# Autodesk Inventor assembly: Frame 1771926384246
(part 2 of 3)
- C:\Users\Admin01\Documents\WU15\TRASTRGNN\Inventor\StructureGenerator\Frame\ANSI UP8 x 30 1771926400178.ipt
- C:\Users\Admin01\Documents\WU15\TRASTRGNN\Inventor\StructureGenerator\Frame\ANSI UP8 x 30 1771926400208.ipt
- C:\Users\Admin01\Documents\WU15\TRASTRGNN\Inventor\StructureGenerator\Frame\ANSI UP8 x 30 1771926400238.ipt
- C:\Users\Admin01\Documents\WU15\TRASTRGNN\Inventor\StructureGenerator\Frame\ANSI UP8 x 30 1771926400267.ipt
- C:\Users\Admin01\Documents\WU15\TRASTRGNN\Inventor\StructureGenerator\Frame\ANSI UP8 x 30 1771926400297.ipt
- C:\Users\Admin01\Documents\WU15\TRASTRGNN\Inventor\StructureGenerator\Frame\ANSI UP8 x 30 1771926400327.ipt
- C:\Users\Admin01\Documents\WU15\TRASTRGNN\Inventor\StructureGenerator\Frame\ANSI UP8 x 30 1771926400356.ipt
- C:\Users\Admin01\Documents\WU15\TRASTRGNN\Inventor\StructureGenerator\Frame\ANSI UP8 x 30 1771926400385.ipt
- C:\Users\Admin01\Documents\WU15\TRASTRGNN\Inventor\StructureGenerator\Frame\ANSI UP8 x 30 1771926400415.ipt
- C:\Users\Admin01\Documents\WU15\TRASTRGNN\Inventor\StructureGenerator\Frame\ANSI UP8 x 30 1771926400444.ipt
- C:\Users\Admin01\Documents\WU15\TRASTRGNN\Inventor\StructureGenerator\Frame\ANSI UP8 x 30 1771926400474.ipt
- C:\Users\Admin01\Documents\WU15\TRASTRGNN\Inventor\StructureGenerator\Frame\ANSI UP8 x 30 1771926400503.ipt
- C:\Users\Admin01\Documents\WU15\TRASTRGNN\Inventor\StructureGenerator\Frame\ANSI UP8 x 30 1771926400533.ipt
- C:\Users\Admin01\Documents\WU15\TRASTRGNN\Inventor\StructureGenerator\Frame\ANSI UP8 x 30 1771926400563.ipt
- C:\Users\Admin01\Documents\WU15\TRASTRGNN\Inventor\StructureGenerator\Frame\ANSI UP8 x 30 1771926400592.ipt
- C:\Users\Admin01\Documents\WU15\TRASTRGNN\Inventor\StructureGenerator\Frame\ANSI UP8 x 30 1771926400622.ipt
- C:\Users\Admin01\Documents\WU15\TRASTRGNN\Inventor\StructureGenerator\Frame\ANSI UP8 x 30 1771926400652.ipt
- C:\Users\Admin01\Documents\WU15\TRASTRGNN\Inventor\StructureGenerator\Frame\ANSI UP8 x 30 1771926400682.ipt
- C:\Users\Admin01\Documents\WU15\TRASTRGNN\Inventor\StructureGenerator\Frame\ANSI UP8 x 30 1771926400712.ipt
- C:\Users\Admin01\Documents\WU15\TRASTRGNN\Inventor\StructureGenerator\Frame\ANSI UP8 x 30 1771926400742.ipt
- C:\Users\Admin01\Documents\WU15\TRASTRGNN\Inventor\StructureGenerator\Frame\ANSI UP8 x 30 1771926400772.ipt
- C:\Users\Admin01\Documents\WU15\TRASTRGNN\Inventor\StructureGenerator\Frame\ANSI UP8 x 30 1771926400801.ipt
- C:\Users\Admin01\Documents\WU15\TRASTRGNN\Inventor\StructureGenerator\Frame\ANSI UP8 x 30 1771926400831.ipt
- C:\Users\Admin01\Documents\WU15\TRASTRGNN\Inventor\StructureGenerator\Frame\ANSI UP8 x 30 1771926400861.ipt
- C:\Users\Admin01\Documents\WU15\TRASTRGNN\Inventor\StructureGenerator\Frame\ANSI UP8 x 30 1771926400890.ipt
- C:\Users\Admin01\Documents\WU15\TRASTRGNN\Inventor\StructureGenerator\Frame\ANSI UP8 x 30 1771926400920.ipt
- C:\Users\Admin01\Documents\WU15\TRASTRGNN\Inventor\StructureGenerator\Frame\ANSI UP8 x 30 1771926400949.ipt
- C:\Users\Admin01\Documents\WU15\TRASTRGNN\Inventor\StructureGenerator\Frame\ANSI UP8 x 30 1771926400979.ipt
- C:\Users\Admin01\Documents\WU15\TRASTRGNN\Inventor\StructureGenerator\Frame\ANSI UP8 x 30 1771926401008.ipt
- C:\Users\Admin01\Documents\WU15\TRASTRGNN\Inventor\StructureGenerator\Frame\ANSI UP8 x 30 1771926401039.ipt
- C:\Users\Admin01\Documents\WU15\TRASTRGNN\Inventor\StructureGenerator\Frame\ANSI UP8 x 30 1771926401068.ipt
- C:\Users\Admin01\Documents\WU15\TRASTRGNN\Inventor\StructureGenerator\Frame\ANSI UP8 x 30 1771926401100.ipt
- C:\Users\Admin01\Documents\WU15\TRASTRGNN\Inventor\StructureGenerator\Frame\ANSI UP8 x 30 1771926401129.ipt
- C:\Users\Admin01\Documents\WU15\TRASTRGNN\Inventor\StructureGenerator\Frame\ANSI UP8 x 30 1771926401159.ipt
- C:\Users\Admin01\Documents\WU15\TRASTRGNN\Inventor\StructureGenerator\Frame\ANSI UP8 x 30 1771926401189.ipt
- C:\Users\Admin01\Documents\WU15\TRASTRGNN\Inventor\StructureGenerator\Frame\ANSI UP8 x 30 1771926401219.ipt
- C:\Users\Admin01\Documents\WU15\TRASTRGNN\Inventor\StructureGenerator\Frame\ANSI UP8 x 30 1771926401248.ipt
- C:\Users\Admin01\Documents\WU15\TRASTRGNN\Inventor\StructureGenerator\Frame\ANSI UP8 x 30 1771926401278.ipt
- C:\Users\Admin01\Documents\WU15\TRASTRGNN\Inventor\StructureGenerator\Frame\ANSI UP8 x 30 1771926401307.ipt
- C:\Users\Admin01\Documents\WU15\TRASTRGNN\Inventor\StructureGenerator\Frame\ANSI UP8 x 30 1771926401337.ipt
- C:\Users\Admin01\Documents\WU15\TRASTRGNN\Inventor\StructureGenerator\Frame\ANSI UP8 x 30 1771926401367.ipt
- C:\Users\Admin01\Documents\WU15\TRASTRGNN\Inventor\StructureGenerator\Frame\ANSI UP8 x 30 1771926401396.ipt
- C:\Users\Admin01\Documents\WU15\TRASTRGNN\Inventor\StructureGenerator\Frame\ANSI UP8 x 30 1771926401425.ipt
- C:\Users\Admin01\Documents\WU15\TRASTRGNN\Inventor\StructureGenerator\Frame\ANSI UP8 x 30 1771926401455.ipt
- C:\Users\Admin01\Documents\WU15\TRASTRGNN\Inventor\StructureGenerator\Frame\ANSI UP8 x 30 1771926401488.ipt
- C:\Users\Admin01\Documents\WU15\TRASTRGNN\Inventor\StructureGenerator\Frame\ANSI UP8 x 30 1771926401519.ipt
- C:\Users\Admin01\Documents\WU15\TRASTRGNN\Inventor\StructureGenerator\Frame\ANSI UP8 x 30 1771926401550.ipt
- C:\Users\Admin01\Documents\WU15\TRASTRGNN\Inventor\StructureGenerator\Frame\ANSI UP8 x 30 1771926401585.ipt
- C:\Users\Admin01\Documents\WU15\TRASTRGNN\Inventor\StructureGenerator\Frame\ANSI UP8 x 30 1771926401618.ipt
- C:\Users\Admin01\Documents\WU15\TRASTRGNN\Inventor\StructureGenerator\Frame\ANSI UP8 x 30 1771926401651.ipt
- C:\Users\Admin01\Documents\WU15\TRASTRGNN\Inventor\StructureGenerator\Frame\ANSI UP8 x 30 1771926401685.ipt
- C:\Users\Admin01\Documents\WU15\TRASTRGNN\Inventor\StructureGenerator\Frame\ANSI UP8 x 30 1771926401716.ipt
- C:\Users\Admin01\Documents\WU15\TRASTRGNN\Inventor\StructureGenerator\Frame\ANSI UP8 x 30 1771926401746.ipt
- C:\Users\Admin01\Documents\WU15\TRASTRGNN\Inventor\StructureGenerator\Frame\ANSI UP8 x 30 1771926401775.ipt
- C:\Users\Admin01\Documents\WU15\TRASTRGNN\Inventor\StructureGenerator\Frame\ANSI UP8 x 30 1771926401805.ipt
- C:\Users\Admin01\Documents\WU15\TRASTRGNN\Inventor\StructureGenerator\Frame\ANSI UP8 x 30 1771926401837.ipt
- C:\Users\Admin01\Documents\WU15\TRASTRGNN\Inventor\StructureGenerator\Frame\ANSI UP8 x 30 1771926401868.ipt
- C:\Users\Admin01\Documents\WU15\TRASTRGNN\Inventor\StructureGenerator\Frame\ANSI UP8 x 30 1771926401898.ipt
- C:\Users\Admin01\Documents\WU15\TRASTRGNN\Inventor\StructureGenerator\Frame\ANSI UP8 x 30 1771926401929.ipt
- C:\Users\Admin01\Documents\WU15\TRASTRGNN\Inventor\StructureGenerator\Frame\ANSI UP8 x 30 1771926401960.ipt
- C:\Users\Admin01\Documents\WU15\TRASTRGNN\Inventor\StructureGenerator\Frame\ANSI UP8 x 30 1771926401992.ipt
- C:\Users\Admin01\Documents\WU15\TRASTRGNN\Inventor\StructureGenerator\Frame\ANSI UP8 x 30 1771926402023.ipt
- C:\Users\Admin01\Documents\WU15\TRASTRGNN\Inventor\StructureGenerator\Frame\ANSI UP8 x 30 1771926402053.ipt
- C:\Users\Admin01\Documents\WU15\TRASTRGNN\Inventor\StructureGenerator\Frame\ANSI UP8 x 30 1771926402084.ipt
- C:\Users\Admin01\Documents\WU15\TRASTRGNN\Inventor\StructureGenerator\Frame\ANSI UP8 x 30 1771926402116.ipt
- C:\Users\Admin01\Documents\WU15\TRASTRGNN\Inventor\StructureGenerator\Frame\ANSI UP8 x 30 1771926402147.ipt
- C:\Users\Admin01\Documents\WU15\TRASTRGNN\Inventor\StructureGenerator\Frame\ANSI UP8 x 30 1771926402182.ipt
- C:\Users\Admin01\Documents\WU15\TRASTRGNN\Inventor\StructureGenerator\Frame\ANSI UP8 x 30 1771926402214.ipt
- C:\Users\Admin01\Documents\WU15\TRASTRGNN\Inventor\StructureGenerator\Frame\ANSI UP8 x 30 1771926402248.ipt
- C:\Users\Admin01\Documents\WU15\TRASTRGNN\Inventor\StructureGenerator\Frame\ANSI UP8 x 30 1771926402278.ipt
- C:\Users\Admin01\Documents\WU15\TRASTRGNN\Inventor\StructureGenerator\Frame\ANSI UP8 x 30 1771926402309.ipt
- C:\Users\Admin01\Documents\WU15\TRASTRGNN\Inventor\StructureGenerator\Frame\ANSI UP8 x 30 1771926402354.ipt
- C:\Users\Admin01\Documents\WU15\TRASTRGNN\Inventor\StructureGenerator\Frame\ANSI UP8 x 30 1771926402386.ipt
- C:\Users\Admin01\Documents\WU15\TRASTRGNN\Inventor\StructureGenerator\Frame\ANSI UP8 x 30 1771926402418.ipt
- C:\Users\Admin01\Documents\WU15\TRASTRGNN\Inventor\StructureGenerator\Frame\ANSI UP8 x 30 1771926402453.ipt
- C:\Users\Admin01\Documents\WU15\TRASTRGNN\Inventor\StructureGenerator\Frame\ANSI UP8 x 30 1771926402485.ipt
- C:\Users\Admin01\Documents\WU15\TRASTRGNN\Inventor\StructureGenerator\Frame\ANSI UP8 x 30 1771926402516.ipt
- C:\Users\Admin01\Documents\WU15\TRASTRGNN\Inventor\StructureGenerator\Frame\ANSI UP8 x 30 1771926402546.ipt
- C:\Users\Admin01\Documents\WU15\TRASTRGNN\Inventor\StructureGenerator\Frame\ANSI UP8 x 30 1771926402576.ipt
- C:\Users\Admin01\Documents\WU15\TRASTRGNN\Inventor\StructureGenerator\Frame\ANSI UP8 x 30 1771926402607.ipt
- C:\Users\Admin01\Documents\WU15\TRASTRGNN\Inventor\StructureGenerator\Frame\ANSI UP8 x 30 1771926402637.ipt
- C:\Users\Admin01\Documents\WU15\TRASTRGNN\Inventor\StructureGenerator\Frame\ANSI UP8 x 30 1771926402667.ipt
- C:\Users\Admin01\Documents\WU15\TRASTRGNN\Inventor\StructureGenerator\Frame\ANSI UP8 x 30 1771926402697.ipt
- C:\Users\Admin01\Documents\WU15\TRASTRGNN\Inventor\StructureGenerator\Frame\ANSI UP8 x 30 1771926402726.ipt
- C:\Users\Admin01\Documents\WU15\TRASTRGNN\Inventor\StructureGenerator\Frame\ANSI UP8 x 30 1771926402756.ipt
- C:\Users\Admin01\Documents\WU15\TRASTRGNN\Inventor\StructureGenerator\Frame\ANSI UP8 x 30 1771926402785.ipt
- C:\Users\Admin01\Documents\WU15\TRASTRGNN\Inventor\StructureGenerator\Frame\ANSI UP8 x 30 1771926402815.ipt
- C:\Users\Admin01\Documents\WU15\TRASTRGNN\Inventor\StructureGenerator\Frame\ANSI UP8 x 30 1771926402844.ipt
- C:\Users\Admin01\Documents\WU15\TRASTRGNN\Inventor\StructureGenerator\Frame\ANSI UP8 x 30 1771926402873.ipt
- C:\Users\Admin01\Documents\WU15\TRASTRGNN\Inventor\StructureGenerator\Frame\ANSI UP8 x 30 1771926402902.ipt
- C:\Users\Admin01\Documents\WU15\TRASTRGNN\Inventor\StructureGenerator\Frame\ANSI UP8 x 30 1771926402932.ipt
- C:\Users\Admin01\Documents\WU15\TRASTRGNN\Inventor\StructureGenerator\Frame\ANSI UP8 x 30 1771926402962.ipt
- C:\Users\Admin01\Documents\WU15\TRASTRGNN\Inventor\StructureGenerator\Frame\ANSI UP8 x 30 1771926402992.ipt
- C:\Users\Admin01\Documents\WU15\TRASTRGNN\Inventor\StructureGenerator\Frame\ANSI UP8 x 30 1771926403021.ipt
- C:\Users\Admin01\Documents\WU15\TRASTRGNN\Inventor\StructureGenerator\Frame\ANSI UP8 x 30 1771926403050.ipt
- C:\Users\Admin01\Documents\WU15\TRASTRGNN\Inventor\StructureGenerator\Frame\ANSI UP8 x 30 1771926403080.ipt
- C:\Users\Admin01\Documents\WU15\TRASTRGNN\Inventor\StructureGenerator\Frame\ANSI UP8 x 30 1771926403110.ipt
- C:\Users\Admin01\Documents\WU15\TRASTRGNN\Inventor\StructureGenerator\Frame\ANSI UP8 x 30 1771926403139.ipt
- C:\Users\Admin01\Documents\WU15\TRASTRGNN\Inventor\StructureGenerator\Frame\ANSI UP8 x 30 1771926403170.ipt
- C:\Users\Admin01\Documents\WU15\TRASTRGNN\Inventor\StructureGenerator\Frame\ANSI UP8 x 30 1771926403200.ipt
- C:\Users\Admin01\Documents\WU15\TRASTRGNN\Inventor\StructureGenerator\Frame\ANSI UP8 x 30 1771926403229.ipt
- C:\Users\Admin01\Documents\WU15\TRASTRGNN\Inventor\StructureGenerator\Frame\ANSI UP8 x 30 1771926403259.ipt
- C:\Users\Admin01\Documents\WU15\TRASTRGNN\Inventor\StructureGenerator\Frame\ANSI UP8 x 30 1771926403289.ipt
- C:\Users\Admin01\Documents\WU15\TRASTRGNN\Inventor\StructureGenerator\Frame\ANSI UP8 x 30 1771926403318.ipt
- C:\Users\Admin01\Documents\WU15\TRASTRGNN\Inventor\StructureGenerator\Frame\ANSI UP8 x 30 1771926403348.ipt
- C:\Users\Admin01\Documents\WU15\TRASTRGNN\Inventor\StructureGenerator\Frame\ANSI UP8 x 30 1771926403378.ipt
- C:\Users\Admin01\Documents\WU15\TRASTRGNN\Inventor\StructureGenerator\Frame\ANSI UP8 x 30 1771926403411.ipt
- C:\Users\Admin01\Documents\WU15\TRASTRGNN\Inventor\StructureGenerator\Frame\ANSI UP8 x 30 1771926403441.ipt
- C:\Users\Admin01\Documents\WU15\TRASTRGNN\Inventor\StructureGenerator\Frame\ANSI UP8 x 30 1771926403470.ipt
- C:\Users\Admin01\Documents\WU15\TRASTRGNN\Inventor\StructureGenerator\Frame\ANSI UP8 x 30 1771926403500.ipt
- C:\Users\Admin01\Documents\WU15\TRASTRGNN\Inventor\StructureGenerator\Frame\ANSI UP8 x 30 1771926403530.ipt
- C:\Users\Admin01\Documents\WU15\TRASTRGNN\Inventor\StructureGenerator\Frame\ANSI UP8 x 30 1771926403560.ipt
- C:\Users\Admin01\Documents\WU15\TRASTRGNN\Inventor\StructureGenerator\Frame\ANSI UP8 x 30 1771926403589.ipt
- C:\Users\Admin01\Documents\WU15\TRASTRGNN\Inventor\StructureGenerator\Frame\ANSI UP8 x 30 1771926403619.ipt
- C:\Users\Admin01\Documents\WU15\TRASTRGNN\Inventor\StructureGenerator\Frame\ANSI UP8 x 30 1771926403648.ipt
- C:\Users\Admin01\Documents\WU15\TRASTRGNN\Inventor\StructureGenerator\Frame\ANSI UP8 x 30 1771926403677.ipt
- C:\Users\Admin01\Documents\WU15\TRASTRGNN\Inventor\StructureGenerator\Frame\ANSI UP8 x 30 1771926403708.ipt
- C:\Users\Admin01\Documents\WU15\TRASTRGNN\Inventor\StructureGenerator\Frame\ANSI UP8 x 30 1771926403737.ipt
- C:\Users\Admin01\Documents\WU15\TRASTRGNN\Inventor\StructureGenerator\Frame\ANSI UP8 x 30 1771926403767.ipt
- C:\Users\Admin01\Documents\WU15\TRASTRGNN\Inventor\StructureGenerator\Frame\ANSI UP8 x 30 1771926403796.ipt
- C:\Users\Admin01\Documents\WU15\TRASTRGNN\Inventor\StructureGenerator\Frame\ANSI UP8 x 30 1771926403825.ipt
- C:\Users\Admin01\Documents\WU15\TRASTRGNN\Inventor\StructureGenerator\Frame\ANSI UP8 x 30 1771926403854.ipt
- C:\Users\Admin01\Documents\WU15\TRASTRGNN\Inventor\StructureGenerator\Frame\ANSI UP8 x 30 1771926403904.ipt
- C:\Users\Admin01\Documents\WU15\TRASTRGNN\Inventor\StructureGenerator\Frame\ANSI UP8 x 30 1771926403933.ipt
- C:\Users\Admin01\Documents\WU15\TRASTRGNN\Inventor\StructureGenerator\Frame\ANSI UP8 x 30 1771926403962.ipt
- C:\Users\Admin01\Documents\WU15\TRASTRGNN\Inventor\StructureGenerator\Frame\ANSI UP8 x 30 1771926403991.ipt
- C:\Users\Admin01\Documents\WU15\TRASTRGNN\Inventor\StructureGenerator\Frame\ANSI UP8 x 30 1771926404020.ipt
- C:\Users\Admin01\Documents\WU15\TRASTRGNN\Inventor\StructureGenerator\Frame\ANSI UP8 x 30 1771926404049.ipt
- C:\Users\Admin01\Documents\WU15\TRASTRGNN\Inventor\StructureGenerator\Frame\ANSI UP8 x 30 1771926404085.ipt
- C:\Users\Admin01\Documents\WU15\TRASTRGNN\Inventor\StructureGenerator\Frame\ANSI UP8 x 30 1771926404114.ipt
- C:\Users\Admin01\Documents\WU15\TRASTRGNN\Inventor\StructureGenerator\Frame\ANSI UP8 x 30 1771926404144.ipt
- C:\Users\Admin01\Documents\WU15\TRASTRGNN\Inventor\StructureGenerator\Frame\ANSI UP8 x 30 1771926404173.ipt
- C:\Users\Admin01\Documents\WU15\TRASTRGNN\Inventor\StructureGenerator\Frame\ANSI UP8 x 30 1771926404203.ipt
- C:\Users\Admin01\Documents\WU15\TRASTRGNN\Inventor\StructureGenerator\Frame\ANSI UP8 x 30 1771926404232.ipt
- C:\Users\Admin01\Documents\WU15\TRASTRGNN\Inventor\StructureGenerator\Frame\ANSI UP8 x 30 1771926404261.ipt
- C:\Users\Admin01\Documents\WU15\TRASTRGNN\Inventor\StructureGenerator\Frame\ANSI UP8 x 30 1771926404291.ipt
- C:\Users\Admin01\Documents\WU15\TRASTRGNN\Inventor\StructureGenerator\Frame\ANSI UP8 x 30 1771926404320.ipt
- C:\Users\Admin01\Documents\WU15\TRASTRGNN\Inventor\StructureGenerator\Frame\ANSI UP8 x 30 1771926404349.ipt
- C:\Users\Admin01\Documents\WU15\TRASTRGNN\Inventor\StructureGenerator\Frame\ANSI UP8 x 30 1771926404379.ipt
- C:\Users\Admin01\Documents\WU15\TRASTRGNN\Inventor\StructureGenerator\Frame\ANSI UP8 x 30 1771926404409.ipt
- C:\Users\Admin01\Documents\WU15\TRASTRGNN\Inventor\StructureGenerator\Frame\ANSI UP8 x 30 1771926404439.ipt
- C:\Users\Admin01\Documents\WU15\TRASTRGNN\Inventor\StructureGenerator\Frame\ANSI UP8 x 30 1771926404470.ipt
- C:\Users\Admin01\Documents\WU15\TRASTRGNN\Inventor\StructureGenerator\Frame\ANSI UP8 x 30 1771926404501.ipt
- C:\Users\Admin01\Documents\WU15\TRASTRGNN\Inventor\StructureGenerator\Frame\ANSI UP8 x 30 1771926404533.ipt
- C:\Users\Admin01\Documents\WU15\TRASTRGNN\Inventor\StructureGenerator\Frame\ANSI UP8 x 30 1771926404563.ipt
- C:\Users\Admin01\Documents\WU15\TRASTRGNN\Inventor\StructureGenerator\Frame\ANSI UP8 x 30 1771926404592.ipt
- C:\Users\Admin01\Documents\WU15\TRASTRGNN\Inventor\StructureGenerator\Frame\ANSI UP8 x 30 1771926404621.ipt
- C:\Users\Admin01\Documents\WU15\TRASTRGNN\Inventor\StructureGenerator\Frame\ANSI UP8 x 30 1771926404651.ipt
- C:\Users\Admin01\Documents\WU15\TRASTRGNN\Inventor\StructureGenerator\Frame\ANSI UP8 x 30 1771926404680.ipt
- C:\Users\Admin01\Documents\WU15\TRASTRGNN\Inventor\StructureGenerator\Frame\ANSI UP8 x 30 1771926404710.ipt
- C:\Users\Admin01\Documents\WU15\TRASTRGNN\Inventor\StructureGenerator\Frame\ANSI UP8 x 30 1771926404740.ipt
- C:\Users\Admin01\Documents\WU15\TRASTRGNN\Inventor\StructureGenerator\Frame\ANSI UP8 x 30 1771926404770.ipt
- C:\Users\Admin01\Documents\WU15\TRASTRGNN\Inventor\StructureGenerator\Frame\ANSI UP8 x 30 1771926404799.ipt
- C:\Users\Admin01\Documents\WU15\TRASTRGNN\Inventor\StructureGenerator\Frame\ANSI UP8 x 30 1771926404829.ipt
- C:\Users\Admin01\Documents\WU15\TRASTRGNN\Inventor\StructureGenerator\Frame\ANSI UP8 x 30 1771926404858.ipt
- C:\Users\Admin01\Documents\WU15\TRASTRGNN\Inventor\StructureGenerator\Frame\ANSI UP8 x 30 1771926404887.ipt
- C:\Users\Admin01\Documents\WU15\TRASTRGNN\Inventor\StructureGenerator\Frame\ANSI UP8 x 30 1771926404916.ipt
- C:\Users\Admin01\Documents\WU15\TRASTRGNN\Inventor\StructureGenerator\Frame\ANSI UP8 x 30 1771926404945.ipt
- C:\Users\Admin01\Documents\WU15\TRASTRGNN\Inventor\StructureGenerator\Frame\ANSI UP8 x 30 1771926404974.ipt
- C:\Users\Admin01\Documents\WU15\TRASTRGNN\Inventor\StructureGenerator\Frame\ANSI UP8 x 30 1771926405002.ipt
- C:\Users\Admin01\Documents\WU15\TRASTRGNN\Inventor\StructureGenerator\Frame\ANSI UP8 x 30 1771926405031.ipt
- C:\Users\Admin01\Documents\WU15\TRASTRGNN\Inventor\StructureGenerator\Frame\ANSI UP8 x 30 1771926405060.ipt
- C:\Users\Admin01\Documents\WU15\TRASTRGNN\Inventor\StructureGenerator\Frame\ANSI UP8 x 30 1771926405089.ipt
- C:\Users\Admin01\Documents\WU15\TRASTRGNN\Inventor\StructureGenerator\Frame\ANSI UP8 x 30 1771926405118.ipt
- C:\Users\Admin01\Documents\WU15\TRASTRGNN\Inventor\StructureGenerator\Frame\ANSI UP8 x 30 1771926405148.ipt
- C:\Users\Admin01\Documents\WU15\TRASTRGNN\Inventor\StructureGenerator\Frame\ANSI UP8 x 30 1771926405177.ipt
- C:\Users\Admin01\Documents\WU15\TRASTRGNN\Inventor\StructureGenerator\Frame\ANSI UP8 x 30 1771926405206.ipt
- C:\Users\Admin01\Documents\WU15\TRASTRGNN\Inventor\StructureGenerator\Frame\ANSI UP8 x 30 1771926405236.ipt
- C:\Users\Admin01\Documents\WU15\TRASTRGNN\Inventor\StructureGenerator\Frame\ANSI UP8 x 30 1771926405266.ipt
- C:\Users\Admin01\Documents\WU15\TRASTRGNN\Inventor\StructureGenerator\Frame\ANSI UP8 x 30 1771926405295.ipt
- C:\Users\Admin01\Documents\WU15\TRASTRGNN\Inventor\StructureGenerator\Frame\ANSI UP8 x 30 1771926405325.ipt
- C:\Users\Admin01\Documents\WU15\TRASTRGNN\Inventor\StructureGenerator\Frame\ANSI UP8 x 30 1771926405355.ipt
- C:\Users\Admin01\Documents\WU15\TRASTRGNN\Inventor\StructureGenerator\Frame\ANSI UP8 x 30 1771926405384.ipt
- C:\Users\Admin01\Documents\WU15\TRASTRGNN\Inventor\StructureGenerator\Frame\ANSI UP8 x 30 1771926405414.ipt
- C:\Users\Admin01\Documents\WU15\TRASTRGNN\Inventor\StructureGenerator\Frame\ANSI UP8 x 30 1771926405444.ipt
- C:\Users\Admin01\Documents\WU15\TRASTRGNN\Inventor\StructureGenerator\Frame\ANSI UP8 x 30 1771926405474.ipt
- C:\Users\Admin01\Documents\WU15\TRASTRGNN\Inventor\StructureGenerator\Frame\ANSI UP8 x 30 1771926405523.ipt
- C:\Users\Admin01\Documents\WU15\TRASTRGNN\Inventor\StructureGenerator\Frame\ANSI UP8 x 30 1771926405555.ipt
- C:\Users\Admin01\Documents\WU15\TRASTRGNN\Inventor\StructureGenerator\Frame\ANSI UP8 x 30 1771926405585.ipt
- C:\Users\Admin01\Documents\WU15\TRASTRGNN\Inventor\StructureGenerator\Frame\ANSI UP8 x 30 1771926405615.ipt
- C:\Users\Admin01\Documents\WU15\TRASTRGNN\Inventor\StructureGenerator\Frame\ANSI UP8 x 30 1771926405647.ipt
- C:\Users\Admin01\Documents\WU15\TRASTRGNN\Inventor\StructureGenerator\Frame\ANSI UP8 x 30 1771926405677.ipt
- C:\Users\Admin01\Documents\WU15\TRASTRGNN\Inventor\StructureGenerator\Frame\ANSI UP8 x 30 1771926405707.ipt
- C:\Users\Admin01\Documents\WU15\TRASTRGNN\Inventor\StructureGenerator\Frame\ANSI UP8 x 30 1771926405749.ipt
- C:\Users\Admin01\Documents\WU15\TRASTRGNN\Inventor\StructureGenerator\Frame\ANSI UP8 x 30 1771926405781.ipt
- C:\Users\Admin01\Documents\WU15\TRASTRGNN\Inventor\StructureGenerator\Frame\ANSI UP8 x 30 1771926405810.ipt
- C:\Users\Admin01\Documents\WU15\TRASTRGNN\Inventor\StructureGenerator\Frame\ANSI UP8 x 30 1771926405840.ipt
- C:\Users\Admin01\Documents\WU15\TRASTRGNN\Inventor\StructureGenerator\Frame\ANSI UP8 x 30 1771926405870.ipt
- C:\Users\Admin01\Documents\WU15\TRASTRGNN\Inventor\StructureGenerator\Frame\ANSI UP8 x 30 1771926405901.ipt
- C:\Users\Admin01\Documents\WU15\TRASTRGNN\Inventor\StructureGenerator\Frame\ANSI UP8 x 30 1771926405931.ipt
- C:\Users\Admin01\Documents\WU15\TRASTRGNN\Inventor\StructureGenerator\Frame\ANSI UP8 x 30 1771926405961.ipt
- C:\Users\Admin01\Documents\WU15\TRASTRGNN\Inventor\StructureGenerator\Frame\ANSI UP8 x 30 1771926405992.ipt
- C:\Users\Admin01\Documents\WU15\TRASTRGNN\Inventor\StructureGenerator\Frame\ANSI UP8 x 30 1771926406022.ipt
- C:\Users\Admin01\Documents\WU15\TRASTRGNN\Inventor\StructureGenerator\Frame\ANSI UP8 x 30 1771926406051.ipt
- C:\Users\Admin01\Documents\WU15\TRASTRGNN\Inventor\StructureGenerator\Frame\ANSI UP8 x 30 1771926406081.ipt
- C:\Users\Admin01\Documents\WU15\TRASTRGNN\Inventor\StructureGenerator\Frame\ANSI UP8 x 30 1771926406110.ipt
- C:\Users\Admin01\Documents\WU15\TRASTRGNN\Inventor\StructureGenerator\Frame\ANSI UP8 x 30 1771926406142.ipt
- C:\Users\Admin01\Documents\WU15\TRASTRGNN\Inventor\StructureGenerator\Frame\ANSI UP8 x 30 1771926406172.ipt
- C:\Users\Admin01\Documents\WU15\TRASTRGNN\Inventor\StructureGenerator\Frame\ANSI UP8 x 30 1771926406202.ipt
- C:\Users\Admin01\Documents\WU15\TRASTRGNN\Inventor\StructureGenerator\Frame\ANSI UP8 x 30 1771926406231.ipt
- C:\Users\Admin01\Documents\WU15\TRASTRGNN\Inventor\StructureGenerator\Frame\ANSI UP8 x 30 1771926406267.ipt
- C:\Users\Admin01\Documents\WU15\TRASTRGNN\Inventor\StructureGenerator\Frame\ANSI UP8 x 30 1771926406297.ipt
- C:\Users\Admin01\Documents\WU15\TRASTRGNN\Inventor\StructureGenerator\Frame\ANSI UP8 x 30 1771926406327.ipt
- C:\Users\Admin01\Documents\WU15\TRASTRGNN\Inventor\StructureGenerator\Frame\ANSI UP8 x 30 1771926406356.ipt
- C:\Users\Admin01\Documents\WU15\TRASTRGNN\Inventor\StructureGenerator\Frame\ANSI UP8 x 30 1771926406385.ipt
- C:\Users\Admin01\Documents\WU15\TRASTRGNN\Inventor\StructureGenerator\Frame\ANSI UP8 x 30 1771926406415.ipt
- C:\Users\Admin01\Documents\WU15\TRASTRGNN\Inventor\StructureGenerator\Frame\ANSI UP8 x 30 1771926406445.ipt
- C:\Users\Admin01\Documents\WU15\TRASTRGNN\Inventor\StructureGenerator\Frame\ANSI UP8 x 30 1771926406475.ipt
- C:\Users\Admin01\Documents\WU15\TRASTRGNN\Inventor\StructureGenerator\Frame\ANSI UP8 x 30 1771926406504.ipt
- C:\Users\Admin01\Documents\WU15\TRASTRGNN\Inventor\StructureGenerator\Frame\ANSI UP8 x 30 1771926406535.ipt
- C:\Users\Admin01\Documents\WU15\TRASTRGNN\Inventor\StructureGenerator\Frame\ANSI UP8 x 30 1771926406564.ipt
- C:\Users\Admin01\Documents\WU15\TRASTRGNN\Inventor\StructureGenerator\Frame\ANSI UP8 x 30 1771926406594.ipt
- C:\Users\Admin01\Documents\WU15\TRASTRGNN\Inventor\StructureGenerator\Frame\ANSI UP8 x 30 1771926406624.ipt
- C:\Users\Admin01\Documents\WU15\TRASTRGNN\Inventor\StructureGenerator\Frame\ANSI UP8 x 30 1771926406653.ipt
- C:\Users\Admin01\Documents\WU15\TRASTRGNN\Inventor\StructureGenerator\Frame\ANSI UP8 x 30 1771926406683.ipt
- C:\Users\Admin01\Documents\WU15\TRASTRGNN\Inventor\StructureGenerator\Frame\ANSI UP8 x 30 1771926406712.ipt
- C:\Users\Admin01\Documents\WU15\TRASTRGNN\Inventor\StructureGenerator\Frame\ANSI UP8 x 30 1771926406742.ipt
- C:\Users\Admin01\Documents\WU15\TRASTRGNN\Inventor\StructureGenerator\Frame\ANSI UP8 x 30 1771926406779.ipt
- C:\Users\Admin01\Documents\WU15\TRASTRGNN\Inventor\StructureGenerator\Frame\ANSI UP8 x 30 1771926406813.ipt
- C:\Users\Admin01\Documents\WU15\TRASTRGNN\Inventor\StructureGenerator\Frame\ANSI UP8 x 30 1771926406844.ipt
- C:\Users\Admin01\Documents\WU15\TRASTRGNN\Inventor\StructureGenerator\Frame\ANSI UP8 x 30 1771926406887.ipt
- C:\Users\Admin01\Documents\WU15\TRASTRGNN\Inventor\StructureGenerator\Frame\ANSI UP8 x 30 1771926406917.ipt
- C:\Users\Admin01\Documents\WU15\TRASTRGNN\Inventor\StructureGenerator\Frame\ANSI UP8 x 30 1771926406951.ipt
- C:\Users\Admin01\Documents\WU15\TRASTRGNN\Inventor\StructureGenerator\Frame\ANSI UP8 x 30 1771926406980.ipt
- C:\Users\Admin01\Documents\WU15\TRASTRGNN\Inventor\StructureGenerator\Frame\ANSI UP8 x 30 1771926407009.ipt
- C:\Users\Admin01\Documents\WU15\TRASTRGNN\Inventor\StructureGenerator\Frame\ANSI UP8 x 30 1771926407043.ipt
- C:\Users\Admin01\Documents\WU15\TRASTRGNN\Inventor\StructureGenerator\Frame\ANSI UP8 x 30 1771926407073.ipt
- C:\Users\Admin01\Documents\WU15\TRASTRGNN\Inventor\StructureGenerator\Frame\ANSI UP8 x 30 1771926407102.ipt
- C:\Users\Admin01\Documents\WU15\TRASTRGNN\Inventor\StructureGenerator\Frame\ANSI UP8 x 30 1771926407131.ipt
- C:\Users\Admin01\Documents\WU15\TRASTRGNN\Inventor\StructureGenerator\Frame\ANSI UP8 x 30 1771926407161.ipt
- C:\Users\Admin01\Documents\WU15\TRASTRGNN\Inventor\StructureGenerator\Frame\ANSI UP8 x 30 1771926407190.ipt
- C:\Users\Admin01\Documents\WU15\TRASTRGNN\Inventor\StructureGenerator\Frame\ANSI UP8 x 30 1771926407220.ipt
- C:\Users\Admin01\Documents\WU15\TRASTRGNN\Inventor\StructureGenerator\Frame\ANSI UP8 x 30 1771926407250.ipt
- C:\Users\Admin01\Documents\WU15\TRASTRGNN\Inventor\StructureGenerator\Frame\ANSI UP8 x 30 1771926407279.ipt
- C:\Users\Admin01\Documents\WU15\TRASTRGNN\Inventor\StructureGenerator\Frame\ANSI UP8 x 30 1771926407308.ipt
- C:\Users\Admin01\Documents\WU15\TRASTRGNN\Inventor\StructureGenerator\Frame\ANSI UP8 x 30 1771926407338.ipt
- C:\Users\Admin01\Documents\WU15\TRASTRGNN\Inventor\StructureGenerator\Frame\ANSI UP8 x 30 1771926407368.ipt
- C:\Users\Admin01\Documents\WU15\TRASTRGNN\Inventor\StructureGenerator\Frame\ANSI UP8 x 30 1771926407397.ipt
- C:\Users\Admin01\Documents\WU15\TRASTRGNN\Inventor\StructureGenerator\Frame\ANSI UP8 x 30 1771926407426.ipt
- C:\Users\Admin01\Documents\WU15\TRASTRGNN\Inventor\StructureGenerator\Frame\ANSI UP8 x 30 1771926407455.ipt
- C:\Users\Admin01\Documents\WU15\TRASTRGNN\Inventor\StructureGenerator\Frame\ANSI UP8 x 30 1771926407486.ipt
- C:\Users\Admin01\Documents\WU15\TRASTRGNN\Inventor\StructureGenerator\Frame\ANSI UP8 x 30 1771926407515.ipt
- C:\Users\Admin01\Documents\WU15\TRASTRGNN\Inventor\StructureGenerator\Frame\ANSI UP8 x 30 1771926407554.ipt
- C:\Users\Admin01\Documents\WU15\TRASTRGNN\Inventor\StructureGenerator\Frame\ANSI UP8 x 30 1771926407584.ipt
- C:\Users\Admin01\Documents\WU15\TRASTRGNN\Inventor\StructureGenerator\Frame\ANSI UP8 x 30 1771926407614.ipt
- C:\Users\Admin01\Documents\WU15\TRASTRGNN\Inventor\StructureGenerator\Frame\ANSI UP8 x 30 1771926407644.ipt
- C:\Users\Admin01\Documents\WU15\TRASTRGNN\Inventor\StructureGenerator\Frame\ANSI UP8 x 30 1771926407674.ipt
- C:\Users\Admin01\Documents\WU15\TRASTRGNN\Inventor\StructureGenerator\Frame\ANSI UP8 x 30 1771926407703.ipt
- C:\Users\Admin01\Documents\WU15\TRASTRGNN\Inventor\StructureGenerator\Frame\ANSI UP8 x 30 1771926407732.ipt
- C:\Users\Admin01\Documents\WU15\TRASTRGNN\Inventor\StructureGenerator\Frame\ANSI UP8 x 30 1771926407762.ipt
- C:\Users\Admin01\Documents\WU15\TRASTRGNN\Inventor\StructureGenerator\Frame\ANSI UP8 x 30 1771926407792.ipt
- C:\Users\Admin01\Documents\WU15\TRASTRGNN\Inventor\StructureGenerator\Frame\ANSI UP8 x 30 1771926407822.ipt
- C:\Users\Admin01\Documents\WU15\TRASTRGNN\Inventor\StructureGenerator\Frame\ANSI UP8 x 30 1771926407852.ipt
- C:\Users\Admin01\Documents\WU15\TRASTRGNN\Inventor\StructureGenerator\Frame\ANSI UP8 x 30 1771926407881.ipt
- C:\Users\Admin01\Documents\WU15\TRASTRGNN\Inventor\StructureGenerator\Frame\ANSI UP8 x 30 1771926407913.ipt
- C:\Users\Admin01\Documents\WU15\TRASTRGNN\Inventor\StructureGenerator\Frame\ANSI UP8 x 30 1771926407942.ipt
- C:\Users\Admin01\Documents\WU15\TRASTRGNN\Inventor\StructureGenerator\Frame\ANSI UP8 x 30 1771926407973.ipt
- C:\Users\Admin01\Documents\WU15\TRASTRGNN\Inventor\StructureGenerator\Frame\ANSI UP8 x 30 1771926408003.ipt
- C:\Users\Admin01\Documents\WU15\TRASTRGNN\Inventor\StructureGenerator\Frame\ANSI UP8 x 30 1771926408033.ipt
- C:\Users\Admin01\Documents\WU15\TRASTRGNN\Inventor\StructureGenerator\Frame\ANSI UP8 x 30 1771926408066.ipt
- C:\Users\Admin01\Documents\WU15\TRASTRGNN\Inventor\StructureGenerator\Frame\ANSI UP8 x 30 1771926408096.ipt
- C:\Users\Admin01\Documents\WU15\TRASTRGNN\Inventor\StructureGenerator\Frame\ANSI UP8 x 30 1771926408126.ipt
- C:\Users\Admin01\Documents\WU15\TRASTRGNN\Inventor\StructureGenerator\Frame\ANSI UP8 x 30 1771926408156.ipt
- C:\Users\Admin01\Documents\WU15\TRASTRGNN\Inventor\StructureGenerator\Frame\ANSI UP8 x 30 1771926408186.ipt
- C:\Users\Admin01\Documents\WU15\TRASTRGNN\Inventor\StructureGenerator\Frame\ANSI UP8 x 30 1771926408216.ipt
- C:\Users\Admin01\Documents\WU15\TRASTRGNN\Inventor\StructureGenerator\Frame\ANSI UP8 x 30 1771926408246.ipt
- C:\Users\Admin01\Documents\WU15\TRASTRGNN\Inventor\StructureGenerator\Frame\ANSI UP8 x 30 1771926408276.ipt
- C:\Users\Admin01\Documents\WU15\TRASTRGNN\Inventor\StructureGenerator\Frame\ANSI UP8 x 30 1771926408306.ipt
- C:\Users\Admin01\Documents\WU15\TRASTRGNN\Inventor\StructureGenerator\Frame\ANSI UP8 x 30 1771926408337.ipt
- C:\Users\Admin01\Documents\WU15\TRASTRGNN\Inventor\StructureGenerator\Frame\ANSI UP8 x 30 1771926408369.ipt
- C:\Users\Admin01\Documents\WU15\TRASTRGNN\Inventor\StructureGenerator\Frame\ANSI UP8 x 30 1771926408400.ipt
- C:\Users\Admin01\Documents\WU15\TRASTRGNN\Inventor\StructureGenerator\Frame\ANSI UP8 x 30 1771926408430.ipt
- C:\Users\Admin01\Documents\WU15\TRASTRGNN\Inventor\StructureGenerator\Frame\ANSI UP8 x 30 1771926408460.ipt
- C:\Users\Admin01\Documents\WU15\TRASTRGNN\Inventor\StructureGenerator\Frame\ANSI UP8 x 30 1771926408490.ipt
- C:\Users\Admin01\Documents\WU15\TRASTRGNN\Inventor\StructureGenerator\Frame\ANSI UP8 x 30 1771926408520.ipt
- C:\Users\Admin01\Documents\WU15\TRASTRGNN\Inventor\StructureGenerator\Frame\ANSI UP8 x 30 1771926408551.ipt
- C:\Users\Admin01\Documents\WU15\TRASTRGNN\Inventor\StructureGenerator\Frame\ANSI UP8 x 30 1771926408581.ipt
- C:\Users\Admin01\Documents\WU15\TRASTRGNN\Inventor\StructureGenerator\Frame\ANSI UP8 x 30 1771926408610.ipt
- C:\Users\Admin01\Documents\WU15\TRASTRGNN\Inventor\StructureGenerator\Frame\ANSI UP8 x 30 1771926408641.ipt
- C:\Users\Admin01\Documents\WU15\TRASTRGNN\Inventor\StructureGenerator\Frame\ANSI UP8 x 30 1771926408671.ipt
- C:\Users\Admin01\Documents\WU15\TRASTRGNN\Inventor\StructureGenerator\Frame\ANSI UP8 x 30 1771926408701.ipt
- C:\Users\Admin01\Documents\WU15\TRASTRGNN\Inventor\StructureGenerator\Frame\ANSI UP8 x 30 1771926408731.ipt
- C:\Users\Admin01\Documents\WU15\TRASTRGNN\Inventor\StructureGenerator\Frame\ANSI UP8 x 30 1771926408760.ipt
- C:\Users\Admin01\Documents\WU15\TRASTRGNN\Inventor\StructureGenerator\Frame\ANSI UP8 x 30 1771926408790.ipt
- C:\Users\Admin01\Documents\WU15\TRASTRGNN\Inventor\StructureGenerator\Frame\ANSI UP8 x 30 1771926408820.ipt
- C:\Users\Admin01\Documents\WU15\TRASTRGNN\Inventor\StructureGenerator\Frame\ANSI UP8 x 30 1771926408850.ipt
- C:\Users\Admin01\Documents\WU15\TRASTRGNN\Inventor\StructureGenerator\Frame\ANSI UP8 x 30 1771926408880.ipt
- C:\Users\Admin01\Documents\WU15\TRASTRGNN\Inventor\StructureGenerator\Frame\ANSI UP8 x 30 1771926408910.ipt
- C:\Users\Admin01\Documents\WU15\TRASTRGNN\Inventor\StructureGenerator\Frame\ANSI UP8 x 30 1771926408940.ipt
- C:\Users\Admin01\Documents\WU15\TRASTRGNN\Inventor\StructureGenerator\Frame\ANSI UP8 x 30 1771926408970.ipt
- C:\Users\Admin01\Documents\WU15\TRASTRGNN\Inventor\StructureGenerator\Frame\ANSI UP8 x 30 1771926409000.ipt
- C:\Users\Admin01\Documents\WU15\TRASTRGNN\Inventor\StructureGenerator\Frame\ANSI UP8 x 30 1771926409032.ipt
- C:\Users\Admin01\Documents\WU15\TRASTRGNN\Inventor\StructureGenerator\Frame\ANSI UP8 x 30 1771926409062.ipt
- C:\Users\Admin01\Documents\WU15\TRASTRGNN\Inventor\StructureGenerator\Frame\ANSI UP8 x 30 1771926409097.ipt
- C:\Users\Admin01\Documents\WU15\TRASTRGNN\Inventor\StructureGenerator\Frame\ANSI UP8 x 30 1771926409128.ipt
- C:\Users\Admin01\Documents\WU15\TRASTRGNN\Inventor\StructureGenerator\Frame\ANSI UP8 x 30 1771926409158.ipt
- C:\Users\Admin01\Documents\WU15\TRASTRGNN\Inventor\StructureGenerator\Frame\ANSI UP8 x 30 1771926409187.ipt
- C:\Users\Admin01\Documents\WU15\TRASTRGNN\Inventor\StructureGenerator\Frame\ANSI UP8 x 30 1771926409217.ipt
- C:\Users\Admin01\Documents\WU15\TRASTRGNN\Inventor\StructureGenerator\Frame\ANSI UP8 x 30 1771926409247.ipt
- C:\Users\Admin01\Documents\WU15\TRASTRGNN\Inventor\StructureGenerator\Frame\ANSI UP8 x 30 1771926409277.ipt
- C:\Users\Admin01\Documents\WU15\TRASTRGNN\Inventor\StructureGenerator\Frame\ANSI UP8 x 30 1771926409314.ipt
- C:\Users\Admin01\Documents\WU15\TRASTRGNN\Inventor\StructureGenerator\Frame\ANSI UP8 x 30 1771926409350.ipt
- C:\Users\Admin01\Documents\WU15\TRASTRGNN\Inventor\StructureGenerator\Frame\ANSI UP8 x 30 1771926409380.ipt
- C:\Users\Admin01\Documents\WU15\TRASTRGNN\Inventor\StructureGenerator\Frame\ANSI UP8 x 30 1771926409410.ipt
- C:\Users\Admin01\Documents\WU15\TRASTRGNN\Inventor\StructureGenerator\Frame\ANSI UP8 x 30 1771926409439.ipt
- C:\Users\Admin01\Documents\WU15\TRASTRGNN\Inventor\StructureGenerator\Frame\ANSI UP8 x 30 1771926409469.ipt
- C:\Users\Admin01\Documents\WU15\TRASTRGNN\Inventor\StructureGenerator\Frame\ANSI UP8 x 30 1771926409499.ipt
- C:\Users\Admin01\Documents\WU15\TRASTRGNN\Inventor\StructureGenerator\Frame\ANSI UP8 x 30 1771926409528.ipt
- C:\Users\Admin01\Documents\WU15\TRASTRGNN\Inventor\StructureGenerator\Frame\ANSI UP8 x 30 1771926409557.ipt
- C:\Users\Admin01\Documents\WU15\TRASTRGNN\Inventor\StructureGenerator\Frame\ANSI UP8 x 30 1771926409587.ipt
- C:\Users\Admin01\Documents\WU15\TRASTRGNN\Inventor\StructureGenerator\Frame\ANSI UP8 x 30 1771926409617.ipt
- C:\Users\Admin01\Documents\WU15\TRASTRGNN\Inventor\StructureGenerator\Frame\ANSI UP8 x 30 1771926409646.ipt
- C:\Users\Admin01\Documents\WU15\TRASTRGNN\Inventor\StructureGenerator\Frame\ANSI UP8 x 30 1771926409676.ipt
- C:\Users\Admin01\Documents\WU15\TRASTRGNN\Inventor\StructureGenerator\Frame\ANSI UP8 x 30 1771926409706.ipt
- C:\Users\Admin01\Documents\WU15\TRASTRGNN\Inventor\StructureGenerator\Frame\ANSI UP8 x 30 1771926409735.ipt
- C:\Users\Admin01\Documents\WU15\TRASTRGNN\Inventor\StructureGenerator\Frame\ANSI UP8 x 30 1771926409765.ipt
- C:\Users\Admin01\Documents\WU15\TRASTRGNN\Inventor\StructureGenerator\Frame\ANSI UP8 x 30 1771926409796.ipt
- C:\Users\Admin01\Documents\WU15\TRASTRGNN\Inventor\StructureGenerator\Frame\ANSI UP8 x 30 1771926409825.ipt
- C:\Users\Admin01\Documents\WU15\TRASTRGNN\Inventor\StructureGenerator\Frame\ANSI UP8 x 30 1771926409855.ipt
- C:\Users\Admin01\Documents\WU15\TRASTRGNN\Inventor\StructureGenerator\Frame\ANSI UP8 x 30 1771926409884.ipt
- C:\Users\Admin01\Documents\WU15\TRASTRGNN\Inventor\StructureGenerator\Frame\ANSI UP8 x 30 1771926409913.ipt
- C:\Users\Admin01\Documents\WU15\TRASTRGNN\Inventor\StructureGenerator\Frame\ANSI UP8 x 30 1771926409943.ipt
- C:\Users\Admin01\Documents\WU15\TRASTRGNN\Inventor\StructureGenerator\Frame\ANSI UP8 x 30 1771926409972.ipt
- C:\Users\Admin01\Documents\WU15\TRASTRGNN\Inventor\StructureGenerator\Frame\ANSI UP8 x 30 1771926410001.ipt
- C:\Users\Admin01\Documents\WU15\TRASTRGNN\Inventor\StructureGenerator\Frame\ANSI UP8 x 30 1771926410031.ipt
- C:\Users\Admin01\Documents\WU15\TRASTRGNN\Inventor\StructureGenerator\Frame\ANSI UP8 x 30 1771926410067.ipt
- C:\Users\Admin01\Documents\WU15\TRASTRGNN\Inventor\StructureGenerator\Frame\ANSI UP8 x 30 1771926410098.ipt
- C:\Users\Admin01\Documents\WU15\TRASTRGNN\Inventor\StructureGenerator\Frame\ANSI UP8 x 30 1771926410130.ipt
- C:\Users\Admin01\Documents\WU15\TRASTRGNN\Inventor\StructureGenerator\Frame\ANSI UP8 x 30 1771926410162.ipt
- C:\Users\Admin01\Documents\WU15\TRASTRGNN\Inventor\StructureGenerator\Frame\ANSI UP8 x 30 1771926410192.ipt
- C:\Users\Admin01\Documents\WU15\TRASTRGNN\Inventor\StructureGenerator\Frame\ANSI UP8 x 30 1771926410222.ipt
- C:\Users\Admin01\Documents\WU15\TRASTRGNN\Inventor\StructureGenerator\Frame\ANSI UP8 x 30 1771926410252.ipt
- C:\Users\Admin01\Documents\WU15\TRASTRGNN\Inventor\StructureGenerator\Frame\ANSI UP8 x 30 1771926410282.ipt
- C:\Users\Admin01\Documents\WU15\TRASTRGNN\Inventor\StructureGenerator\Frame\ANSI UP8 x 30 1771926410312.ipt
- C:\Users\Admin01\Documents\WU15\TRASTRGNN\Inventor\StructureGenerator\Frame\ANSI UP8 x 30 1771926410341.ipt
- C:\Users\Admin01\Documents\WU15\TRASTRGNN\Inventor\StructureGenerator\Frame\ANSI UP8 x 30 1771926410371.ipt
- C:\Users\Admin01\Documents\WU15\TRASTRGNN\Inventor\StructureGenerator\Frame\ANSI UP8 x 30 1771926410401.ipt
- C:\Users\Admin01\Documents\WU15\TRASTRGNN\Inventor\StructureGenerator\Frame\ANSI UP8 x 30 1771926410430.ipt
- C:\Users\Admin01\Documents\WU15\TRASTRGNN\Inventor\StructureGenerator\Frame\ANSI UP8 x 30 1771926410459.ipt
- C:\Users\Admin01\Documents\WU15\TRASTRGNN\Inventor\StructureGenerator\Frame\ANSI UP8 x 30 1771926410489.ipt
- C:\Users\Admin01\Documents\WU15\TRASTRGNN\Inventor\StructureGenerator\Frame\ANSI UP8 x 30 1771926410519.ipt
- C:\Users\Admin01\Documents\WU15\TRASTRGNN\Inventor\StructureGenerator\Frame\ANSI UP8 x 30 1771926410549.ipt
- C:\Users\Admin01\Documents\WU15\TRASTRGNN\Inventor\StructureGenerator\Frame\ANSI UP8 x 30 1771926410578.ipt
- C:\Users\Admin01\Documents\WU15\TRASTRGNN\Inventor\StructureGenerator\Frame\ANSI UP8 x 30 1771926410609.ipt
- C:\Users\Admin01\Documents\WU15\TRASTRGNN\Inventor\StructureGenerator\Frame\ANSI UP8 x 30 1771926410640.ipt
- C:\Users\Admin01\Documents\WU15\TRASTRGNN\Inventor\StructureGenerator\Frame\ANSI UP8 x 30 1771926410674.ipt
- C:\Users\Admin01\Documents\WU15\TRASTRGNN\Inventor\StructureGenerator\Frame\ANSI UP8 x 30 1771926410706.ipt
- C:\Users\Admin01\Documents\WU15\TRASTRGNN\Inventor\StructureGenerator\Frame\ANSI UP8 x 30 1771926410739.ipt
- C:\Users\Admin01\Documents\WU15\TRASTRGNN\Inventor\StructureGenerator\Frame\ANSI UP8 x 30 1771926410769.ipt
- C:\Users\Admin01\Documents\WU15\TRASTRGNN\Inventor\StructureGenerator\Frame\ANSI UP8 x 30 1771926410798.ipt
- C:\Users\Admin01\Documents\WU15\TRASTRGNN\Inventor\StructureGenerator\Frame\ANSI UP8 x 30 1771926410829.ipt
- C:\Users\Admin01\Documents\WU15\TRASTRGNN\Inventor\StructureGenerator\Frame\ANSI UP8 x 30 1771926410858.ipt
- C:\Users\Admin01\Documents\WU15\TRASTRGNN\Inventor\StructureGenerator\Frame\ANSI UP8 x 30 1771926410888.ipt
- C:\Users\Admin01\Documents\WU15\TRASTRGNN\Inventor\StructureGenerator\Frame\ANSI UP8 x 30 1771926410918.ipt
- C:\Users\Admin01\Documents\WU15\TRASTRGNN\Inventor\StructureGenerator\Frame\ANSI UP8 x 30 1771926410948.ipt
- C:\Users\Admin01\Documents\WU15\TRASTRGNN\Inventor\StructureGenerator\Frame\ANSI UP8 x 30 1771926410977.ipt
- C:\Users\Admin01\Documents\WU15\TRASTRGNN\Inventor\StructureGenerator\Frame\ANSI UP8 x 30 1771926411007.ipt
- C:\Users\Admin01\Documents\WU15\TRASTRGNN\Inventor\StructureGenerator\Frame\ANSI UP8 x 30 1771926411036.ipt
- C:\Users\Admin01\Documents\WU15\TRASTRGNN\Inventor\StructureGenerator\Frame\ANSI UP8 x 30 1771926411065.ipt
- C:\Users\Admin01\Documents\WU15\TRASTRGNN\Inventor\StructureGenerator\Frame\ANSI UP8 x 30 1771926411095.ipt
- C:\Users\Admin01\Documents\WU15\TRASTRGNN\Inventor\StructureGenerator\Frame\ANSI UP8 x 30 1771926411124.ipt
- C:\Users\Admin01\Documents\WU15\TRASTRGNN\Inventor\StructureGenerator\Frame\ANSI UP8 x 30 1771926411153.ipt
- C:\Users\Admin01\Documents\WU15\TRASTRGNN\Inventor\StructureGenerator\Frame\ANSI UP8 x 30 1771926411184.ipt
- C:\Users\Admin01\Documents\WU15\TRASTRGNN\Inventor\StructureGenerator\Frame\ANSI UP8 x 30 1771926411214.ipt
- C:\Users\Admin01\Documents\WU15\TRASTRGNN\Inventor\StructureGenerator\Frame\ANSI UP8 x 30 1771926411244.ipt
- C:\Users\Admin01\Documents\WU15\TRASTRGNN\Inventor\StructureGenerator\Frame\ANSI UP8 x 30 1771926411277.ipt
- C:\Users\Admin01\Documents\WU15\TRASTRGNN\Inventor\StructureGenerator\Frame\ANSI UP8 x 30 1771926411307.ipt
- C:\Users\Admin01\Documents\WU15\TRASTRGNN\Inventor\StructureGenerator\Frame\ANSI UP8 x 30 1771926411338.ipt
- C:\Users\Admin01\Documents\WU15\TRASTRGNN\Inventor\StructureGenerator\Frame\ANSI UP8 x 30 1771926411373.ipt
- C:\Users\Admin01\Documents\WU15\TRASTRGNN\Inventor\StructureGenerator\Frame\ANSI UP8 x 30 1771926411403.ipt
- C:\Users\Admin01\Documents\WU15\TRASTRGNN\Inventor\StructureGenerator\Frame\ANSI UP8 x 30 1771926411433.ipt
- C:\Users\Admin01\Documents\WU15\TRASTRGNN\Inventor\StructureGenerator\Frame\ANSI UP8 x 30 1771926411465.ipt
- C:\Users\Admin01\Documents\WU15\TRASTRGNN\Inventor\StructureGenerator\Frame\ANSI UP8 x 30 1771926411495.ipt
- C:\Users\Admin01\Documents\WU15\TRASTRGNN\Inventor\StructureGenerator\Frame\ANSI UP8 x 30 1771926411525.ipt
- C:\Users\Admin01\Documents\WU15\TRASTRGNN\Inventor\StructureGenerator\Frame\ANSI UP8 x 30 1771926411555.ipt
- C:\Users\Admin01\Documents\WU15\TRASTRGNN\Inventor\StructureGenerator\Frame\ANSI UP8 x 30 1771926411585.ipt
- C:\Users\Admin01\Documents\WU15\TRASTRGNN\Inventor\StructureGenerator\Frame\ANSI UP8 x 30 1771926411615.ipt
- C:\Users\Admin01\Documents\WU15\TRASTRGNN\Inventor\StructureGenerator\Frame\ANSI UP8 x 30 1771926411645.ipt
- C:\Users\Admin01\Documents\WU15\TRASTRGNN\Inventor\StructureGenerator\Frame\ANSI UP8 x 30 1771926411674.ipt
- C:\Users\Admin01\Documents\WU15\TRASTRGNN\Inventor\StructureGenerator\Frame\ANSI UP8 x 30 1771926411704.ipt
- C:\Users\Admin01\Documents\WU15\TRASTRGNN\Inventor\StructureGenerator\Frame\ANSI UP8 x 30 1771926411734.ipt
- C:\Users\Admin01\Documents\WU15\TRASTRGNN\Inventor\StructureGenerator\Frame\ANSI UP8 x 30 1771926411763.ipt
- C:\Users\Admin01\Documents\WU15\TRASTRGNN\Inventor\StructureGenerator\Frame\ANSI UP8 x 30 1771926411793.ipt
- C:\Users\Admin01\Documents\WU15\TRASTRGNN\Inventor\StructureGenerator\Frame\ANSI UP8 x 30 1771926411822.ipt
- C:\Users\Admin01\Documents\WU15\TRASTRGNN\Inventor\StructureGenerator\Frame\ANSI UP8 x 30 1771926411852.ipt
- C:\Users\Admin01\Documents\WU15\TRASTRGNN\Inventor\StructureGenerator\Frame\ANSI UP8 x 30 1771926411881.ipt
- C:\Users\Admin01\Documents\WU15\TRASTRGNN\Inventor\StructureGenerator\Frame\ANSI UP8 x 30 1771926411911.ipt
- C:\Users\Admin01\Documents\WU15\TRASTRGNN\Inventor\StructureGenerator\Frame\ANSI UP8 x 30 1771926411940.ipt
- C:\Users\Admin01\Documents\WU15\TRASTRGNN\Inventor\StructureGenerator\Frame\ANSI UP8 x 30 1771926411970.ipt
- C:\Users\Admin01\Documents\WU15\TRASTRGNN\Inventor\StructureGenerator\Frame\ANSI UP8 x 30 1771926411999.ipt
- C:\Users\Admin01\Documents\WU15\TRASTRGNN\Inventor\StructureGenerator\Frame\ANSI UP8 x 30 1771926412028.ipt
- C:\Users\Admin01\Documents\WU15\TRASTRGNN\Inventor\StructureGenerator\Frame\ANSI UP8 x 30 1771926412058.ipt
- C:\Users\Admin01\Documents\WU15\TRASTRGNN\Inventor\StructureGenerator\Frame\ANSI UP8 x 30 1771926412087.ipt
## Components (841 placed, 3 different names)
1. Reference Skeleton
2. ANSI UP8 x 30 - 81.102:1
3. ANSI UP8 x 30 - 81.102:2
4. ANSI UP8 x 30 - 125.591:1
5. ANSI UP8 x 30 - 81.102:3
6. ANSI UP8 x 30 - 125.591:2
7. ANSI UP8 x 30 - 81.102:4
8. ANSI UP8 x 30 - 81.102:5
9. ANSI UP8 x 30 - 125.591:3
10. ANSI UP8 x 30 - 125.591:4
11. ANSI UP8 x 30 - 125.591:5
12. ANSI UP8 x 30 - 125.591:6
13. ANSI UP8 x 30 - 81.102:6
14. ANSI UP8 x 30 - 81.102:7
15. ANSI UP8 x 30 - 81.102:8
16. ANSI UP8 x 30 - 125.591:7
17. ANSI UP8 x 30 - 125.591:8
18. ANSI UP8 x 30 - 81.102:9
19. ANSI UP8 x 30 - 81.102:10
20. ANSI UP8 x 30 - 125.591:9
21. ANSI UP8 x 30 - 125.591:10
22. ANSI UP8 x 30 - 81.102:11
23. ANSI UP8 x 30 - 125.591:11
24. ANSI UP8 x 30 - 125.591:12
25. ANSI UP8 x 30 - 125.591:13
26. ANSI UP8 x 30 - 125.591:14
27. ANSI UP8 x 30 - 81.102:12
28. ANSI UP8 x 30 - 125.591:15
29. ANSI UP8 x 30 - 125.591:16
30. ANSI UP8 x 30 - 81.102:13
31. ANSI UP8 x 30 - 81.102:14
32. ANSI UP8 x 30 - 125.591:17
33. ANSI UP8 x 30 - 125.591:18
34. ANSI UP8 x 30 - 81.102:15
35. ANSI UP8 x 30 - 125.591:19
36. ANSI UP8 x 30 - 125.591:20
37. ANSI UP8 x 30 - 81.102:16
38. ANSI UP8 x 30 - 81.102:17
39. ANSI UP8 x 30 - 81.102:18
40. ANSI UP8 x 30 - 125.591:21
41. ANSI UP8 x 30 - 125.591:22
42. ANSI UP8 x 30 - 125.591:23
43. ANSI UP8 x 30 - 125.591:24
44. ANSI UP8 x 30 - 125.591:25
45. ANSI UP8 x 30 - 81.102:19
46. ANSI UP8 x 30 - 125.591:26
47. ANSI UP8 x 30 - 125.591:27
48. ANSI UP8 x 30 - 81.102:20
49. ANSI UP8 x 30 - 125.591:28
50. ANSI UP8 x 30 - 81.102:21
51. ANSI UP8 x 30 - 125.591:29
52. ANSI UP8 x 30 - 125.591:30
53. ANSI UP8 x 30 - 125.591:31
54. ANSI UP8 x 30 - 125.591:32
55. ANSI UP8 x 30 - 125.591:33
56. ANSI UP8 x 30 - 81.102:22
57. ANSI UP8 x 30 - 125.591:34
58. ANSI UP8 x 30 - 81.102:23
59. ANSI UP8 x 30 - 81.102:24
60. ANSI UP8 x 30 - 81.102:25
61. ANSI UP8 x 30 - 125.591:35
62. ANSI UP8 x 30 - 125.591:36
63. ANSI UP8 x 30 - 81.102:26
64. ANSI UP8 x 30 - 125.591:37
65. ANSI UP8 x 30 - 125.591:38
66. ANSI UP8 x 30 - 81.102:27
67. ANSI UP8 x 30 - 81.102:28
68. ANSI UP8 x 30 - 81.102:29
69. ANSI UP8 x 30 - 125.591:39
70. ANSI UP8 x 30 - 125.591:40
71. ANSI UP8 x 30 - 125.591:41
72. ANSI UP8 x 30 - 125.591:42
73. ANSI UP8 x 30 - 125.591:43
74. ANSI UP8 x 30 - 125.591:44
75. ANSI UP8 x 30 - 125.591:45
76. ANSI UP8 x 30 - 125.591:46
77. ANSI UP8 x 30 - 81.102:30
78. ANSI UP8 x 30 - 125.591:47
79. ANSI UP8 x 30 - 125.591:48
80. ANSI UP8 x 30 - 81.102:31
81. ANSI UP8 x 30 - 125.591:49
82. ANSI UP8 x 30 - 125.591:50
83. ANSI UP8 x 30 - 81.102:32
84. ANSI UP8 x 30 - 125.591:51
85. ANSI UP8 x 30 - 125.591:52
86. ANSI UP8 x 30 - 125.591:53
87. ANSI UP8 x 30 - 81.102:33
88. ANSI UP8 x 30 - 125.591:54
89. ANSI UP8 x 30 - 81.102:34
90. ANSI UP8 x 30 - 81.102:35
91. ANSI UP8 x 30 - 125.591:55
92. ANSI UP8 x 30 - 125.591:56
93. ANSI UP8 x 30 - 81.102:36
94. ANSI UP8 x 30 - 81.102:37
95. ANSI UP8 x 30 - 125.591:57
96. ANSI UP8 x 30 - 125.591:58
97. ANSI UP8 x 30 - 81.102:38
98. ANSI UP8 x 30 - 125.591:59
99. ANSI UP8 x 30 - 125.591:60
100. ANSI UP8 x 30 - 81.102:39
101. ANSI UP8 x 30 - 81.102:40
102. ANSI UP8 x 30 - 125.591:61
103. ANSI UP8 x 30 - 81.102:41
104. ANSI UP8 x 30 - 125.591:62
105. ANSI UP8 x 30 - 81.102:42
106. ANSI UP8 x 30 - 81.102:43
107. ANSI UP8 x 30 - 125.591:63
108. ANSI UP8 x 30 - 125.591:64
109. ANSI UP8 x 30 - 125.591:65
110. ANSI UP8 x 30 - 125.591:66
111. ANSI UP8 x 30 - 125.591:67
112. ANSI UP8 x 30 - 125.591:68
113. ANSI UP8 x 30 - 125.591:69
114. ANSI UP8 x 30 - 125.591:70
115. ANSI UP8 x 30 - 125.591:71
116. ANSI UP8 x 30 - 81.102:44
117. ANSI UP8 x 30 - 125.591:72
118. ANSI UP8 x 30 - 81.102:45
119. ANSI UP8 x 30 - 125.591:73
120. ANSI UP8 x 30 - 125.591:74
121. ANSI UP8 x 30 - 125.591:75
122. ANSI UP8 x 30 - 125.591:76
123. ANSI UP8 x 30 - 81.102:46
124. ANSI UP8 x 30 - 125.591:77
125. ANSI UP8 x 30 - 81.102:47
126. ANSI UP8 x 30 - 125.591:78
127. ANSI UP8 x 30 - 125.591:79
128. ANSI UP8 x 30 - 125.591:80
129. ANSI UP8 x 30 - 125.591:81
130. ANSI UP8 x 30 - 81.102:48
131. ANSI UP8 x 30 - 125.591:82
132. ANSI UP8 x 30 - 81.102:49
133. ANSI UP8 x 30 - 81.102:50
134. ANSI UP8 x 30 - 125.591:83
135. ANSI UP8 x 30 - 125.591:84
136. ANSI UP8 x 30 - 81.102:51
137. ANSI UP8 x 30 - 81.102:52
138. ANSI UP8 x 30 - 125.591:85
139. ANSI UP8 x 30 - 125.591:86
140. ANSI UP8 x 30 - 81.102:53
141. ANSI UP8 x 30 - 125.591:87
142. ANSI UP8 x 30 - 81.102:54
143. ANSI UP8 x 30 - 81.102:55
144. ANSI UP8 x 30 - 81.102:56
145. ANSI UP8 x 30 - 125.591:88
146. ANSI UP8 x 30 - 125.591:89
147. ANSI UP8 x 30 - 81.102:57
148. ANSI UP8 x 30 - 81.102:58
149. ANSI UP8 x 30 - 125.591:90
150. ANSI UP8 x 30 - 125.591:91
151. ANSI UP8 x 30 - 81.102:59
152. ANSI UP8 x 30 - 81.102:60
153. ANSI UP8 x 30 - 125.591:92
154. ANSI UP8 x 30 - 125.591:93
155. ANSI UP8 x 30 - 125.591:94
156. ANSI UP8 x 30 - 125.591:95
157. ANSI UP8 x 30 - 125.591:96
158. ANSI UP8 x 30 - 125.591:97
159. ANSI UP8 x 30 - 125.591:98
160. ANSI UP8 x 30 - 125.591:99
161. ANSI UP8 x 30 - 125.591:100
162. ANSI UP8 x 30 - 125.591:101
163. ANSI UP8 x 30 - 125.591:102
164. ANSI UP8 x 30 - 81.102:61
165. ANSI UP8 x 30 - 125.591:103
166. ANSI UP8 x 30 - 81.102:62
167. ANSI UP8 x 30 - 125.591:104
168. ANSI UP8 x 30 - 125.591:105
169. ANSI UP8 x 30 - 125.591:106
170. ANSI UP8 x 30 - 125.591:107
171. ANSI UP8 x 30 - 81.102:63
172. ANSI UP8 x 30 - 125.591:108
173. ANSI UP8 x 30 - 81.102:64
174. ANSI UP8 x 30 - 125.591:109
175. ANSI UP8 x 30 - 81.102:65
176. ANSI UP8 x 30 - 125.591:110
177. ANSI UP8 x 30 - 125.591:111
178. ANSI UP8 x 30 - 125.591:112
179. ANSI UP8 x 30 - 81.102:66
180. ANSI UP8 x 30 - 125.591:113
181. ANSI UP8 x 30 - 125.591:114
182. ANSI UP8 x 30 - 81.102:67
183. ANSI UP8 x 30 - 81.102:68
184. ANSI UP8 x 30 - 125.591:115
185. ANSI UP8 x 30 - 125.591:116
186. ANSI UP8 x 30 - 81.102:69
187. ANSI UP8 x 30 - 125.591:117
188. ANSI UP8 x 30 - 125.591:118
189. ANSI UP8 x 30 - 81.102:70
190. ANSI UP8 x 30 - 81.102:71
191. ANSI UP8 x 30 - 125.591:119
192. ANSI UP8 x 30 - 81.102:72
193. ANSI UP8 x 30 - 125.591:120
194. ANSI UP8 x 30 - 125.591:121
195. ANSI UP8 x 30 - 81.102:73
196. ANSI UP8 x 30 - 81.102:74
197. ANSI UP8 x 30 - 125.591:122
198. ANSI UP8 x 30 - 81.102:75
199. ANSI UP8 x 30 - 81.102:76
200. ANSI UP8 x 30 - 125.591:123
201. ANSI UP8 x 30 - 125.591:124
202. ANSI UP8 x 30 - 81.102:77
203. ANSI UP8 x 30 - 81.102:78
204. ANSI UP8 x 30 - 125.591:125
205. ANSI UP8 x 30 - 125.591:126
206. ANSI UP8 x 30 - 125.591:127
207. ANSI UP8 x 30 - 125.591:128
208. ANSI UP8 x 30 - 125.591:129
209. ANSI UP8 x 30 - 125.591:130
210. ANSI UP8 x 30 - 125.591:131
211. ANSI UP8 x 30 - 125.591:132